# Autodesk Inventor assembly: 10-SUSP-PROFILE-02
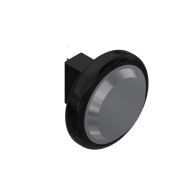
[picture p0: Inventor's stored thumbnail of the model, 180x180]
Saved by Autodesk Inventor 2018.1 (Build 221171000, 171)
## iProperties
Created: 2017-08-13
Part Number: 10-SUSP-PROFILE-02
Document SubType Name: Assembly
Designer: feesmrt
Author: feesmrt
## Documents named in this file (3)
- C:\Users\feesmrt\Documents\NRBDL\Inventor-NRBDL\10-SUSP\10-SUSP-PROFILE-02.iam
- C:\Users\feesmrt\Documents\NRBDL\Inventor-NRBDL\10-SUSP\10-SUSP-03.iam
- C:\Users\feesmrt\Documents\NRBDL\Inventor-NRBDL\20-CASE\WINKEL_30X30_NO_SCREWS.ipt
## Components (3 placed, 2 different names)
1. 10-SUSP-03:1 [sub-assembly] — Fluchtend:1, Passend:2, Fluchtend:4, Fluchtend:5, Passend:3, Fluchtend:6, Fluchtend:7
2. WINKEL_30X30_NO_SCREWS:1 — Fluchtend:1, Fluchtend:5, Passend:3, Fluchtend:6
3. WINKEL_30X30_NO_SCREWS:2 — Passend:2, Fluchtend:4, Fluchtend:7
## Relationships (7: Flush 5, Mate 2)
- Fluchtend:1 [Flush]: 10-SUSP-03:1 ↔ WINKEL_30X30_NO_SCREWS:1
- Passend:2 [Mate]: 10-SUSP-03:1 ↔ WINKEL_30X30_NO_SCREWS:2
- Fluchtend:4 [Flush]: 10-SUSP-03:1 ↔ WINKEL_30X30_NO_SCREWS:2
- Fluchtend:5 [Flush] (16 mm): 10-SUSP-03:1 ↔ WINKEL_30X30_NO_SCREWS:1
- Passend:3 [Mate]: 10-SUSP-03:1 ↔ WINKEL_30X30_NO_SCREWS:1
- Fluchtend:6 [Flush]: 10-SUSP-03:1 ↔ WINKEL_30X30_NO_SCREWS:1
- Fluchtend:7 [Flush]: 10-SUSP-03:1 ↔ WINKEL_30X30_NO_SCREWS:2
